# Autodesk Inventor assembly: BevelTo20TSpureGear
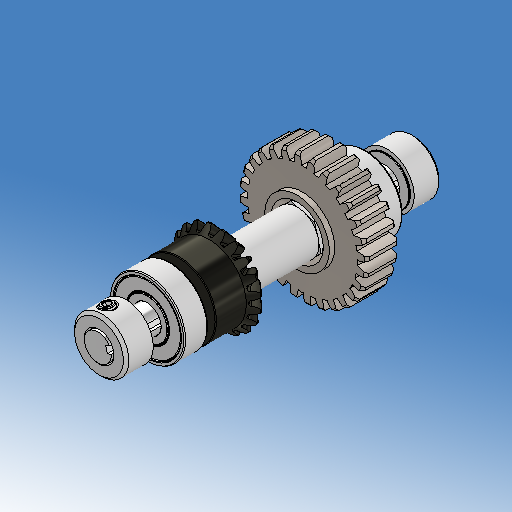
[picture p0: Inventor's stored thumbnail of the model, 512x512]
Saved by Autodesk Inventor 2025 (Build 290162000, 162)
## iProperties
Created: 2024-04-23
Part Number: BevelTo20TSpureGear
Document SubType Name: Assembly
Designer: seene
Author: seene
## Documents named in this file (11)
- C:\Users\seene\OneDrive\SBRT\Robocup Rescue\Drive\v1\BevelTo20TSpureGear.iam
- C:\Users\seene\OneDrive\SBRT\Robocup Rescue\Drive\v1\1439K211_1045 Carbon Steel Keyed Rotary Shaft.ipt
- C:\Users\seene\OneDrive\SBRT\Robocup Rescue\Drive\v1\am-3776 Miter Gear 1.25, 20T, 8mm, 2mm Key Bore.ipt
- C:\Users\seene\OneDrive\SBRT\Robocup Rescue\Drive\v1\am-0588_short 8mm 500 Hex Adapter Shaft 500 long.ipt
- C:\Users\seene\OneDrive\SBRT\Robocup Rescue\Drive\v1\Gears\am-5133 28T 20DP 500hex 375 FW.ipt
- C:\Users\seene\OneDrive\SBRT\Robocup Rescue\Drive\v1\2349K744_Permanently Lubricated Ball Bearing.ipt
- C:\Users\seene\OneDrive\SBRT\Robocup Rescue\Drive\v1\8mKeyyedShaftSpacer_BevelToSpurShaft.ipt
- C:\Users\seene\OneDrive\SBRT\Robocup Rescue\Drive\v1\MachinedKeyStock_BevelToSpur.ipt
- C:\Users\seene\OneDrive\SBRT\Robocup Rescue\Drive\v1\8mmKeyedShaftLongSpacer_BevelToSpurShaft.ipt
- C:\Users\seene\OneDrive\SBRT\Robocup Rescue\Drive\v1\98089A336_18-8 Stainless Steel Round Shim.ipt
- C:\Users\seene\OneDrive\SBRT\Robocup Rescue\Drive\v1\6056N16_Carbon Steel Set Screw Collar.ipt
## Components (14 placed, 10 different names)
1. 1439K211_1045 Carbon Steel Keyed Rotary Shaft:1 — Mate:26, Mate:27, Mate:29, Mate:30, Mate:31, Mate:32, Mate:33, Mate:34, Mate:35, Mate:36, Mate:37, Mate:38, Mate:39, Mate:41
2. am-3776 Miter Gear 1.25, 20T, 8mm, 2mm Key Bore:1 — Mate:19, Flush:8, Mate:22, Flush:9, Flush:10
3. am-0588_short 8mm 500 Hex Adapter Shaft 500 long:1 — Mate:4, Mate:32, Flush:11
4. am-5133 28T 20DP 500hex 375 FW:1 — Mate:4, Mate:25, Mate:33, Flush:11
5. 2349K744_Permanently Lubricated Ball Bearing:1 — Mate:11, Mate:17, Mate:35, Flush:14
6. 2349K744_Permanently Lubricated Ball Bearing:2 — Mate:11, Mate:23, Mate:26, Mate:27, Mate:28, Flush:15
7. 8mKeyyedShaftSpacer_BevelToSpurShaft:1 — Mate:17, Mate:19, Mate:36
8. MachinedKeyStock_BevelToSpur:1 — Flush:8, Mate:30, Mate:31
9. 8mmKeyedShaftLongSpacer_BevelToSpurShaft:1 — Mate:22, Flush:9, Flush:10, Mate:34
10. 98089A336_18-8 Stainless Steel Round Shim:1 — Mate:23, Mate:25, Mate:28, Mate:29
11. 6056N16_Carbon Steel Set Screw Collar:1 — Mate:37, Mate:40
12. 6056N16_Carbon Steel Set Screw Collar:2 — Mate:38, Mate:42
13. 98089A336_18-8 Stainless Steel Round Shim:2 — Mate:39, Flush:14, Mate:40
14. 98089A336_18-8 Stainless Steel Round Shim:3 — Mate:41, Flush:15, Mate:42
## Relationships (30: Mate 24, Flush 6)
- Mate:4: am-0588_short 8mm 500 Hex Adapter Shaft 500 long:1 ↔ am-5133 28T 20DP 500hex 375 FW:1
- Mate:11 (50.8 mm): 2349K744_Permanently Lubricated Ball Bearing:1 ↔ 2349K744_Permanently Lubricated Ball Bearing:2
- Mate:17: 2349K744_Permanently Lubricated Ball Bearing:1 ↔ 8mKeyyedShaftSpacer_BevelToSpurShaft:1
- Mate:19: am-3776 Miter Gear 1.25, 20T, 8mm, 2mm Key Bore:1 ↔ 8mKeyyedShaftSpacer_BevelToSpurShaft:1
- Flush:8: am-3776 Miter Gear 1.25, 20T, 8mm, 2mm Key Bore:1 ↔ MachinedKeyStock_BevelToSpur:1
- Mate:22: am-3776 Miter Gear 1.25, 20T, 8mm, 2mm Key Bore:1 ↔ 8mmKeyedShaftLongSpacer_BevelToSpurShaft:1
- Flush:9: am-3776 Miter Gear 1.25, 20T, 8mm, 2mm Key Bore:1 ↔ 8mmKeyedShaftLongSpacer_BevelToSpurShaft:1
- Flush:10: am-3776 Miter Gear 1.25, 20T, 8mm, 2mm Key Bore:1 ↔ 8mmKeyedShaftLongSpacer_BevelToSpurShaft:1
- Mate:23: 2349K744_Permanently Lubricated Ball Bearing:2 ↔ 98089A336_18-8 Stainless Steel Round Shim:1
- Mate:25: am-5133 28T 20DP 500hex 375 FW:1 ↔ 98089A336_18-8 Stainless Steel Round Shim:1
- Mate:26 (-21.2 mm): 1439K211_1045 Carbon Steel Keyed Rotary Shaft:1 ↔ 2349K744_Permanently Lubricated Ball Bearing:2
- Mate:27: 1439K211_1045 Carbon Steel Keyed Rotary Shaft:1 ↔ 2349K744_Permanently Lubricated Ball Bearing:2
- Mate:28: 2349K744_Permanently Lubricated Ball Bearing:2 ↔ 98089A336_18-8 Stainless Steel Round Shim:1
- Mate:29: 1439K211_1045 Carbon Steel Keyed Rotary Shaft:1 ↔ 98089A336_18-8 Stainless Steel Round Shim:1
- Mate:30: 1439K211_1045 Carbon Steel Keyed Rotary Shaft:1 ↔ MachinedKeyStock_BevelToSpur:1
- Mate:31: 1439K211_1045 Carbon Steel Keyed Rotary Shaft:1 ↔ MachinedKeyStock_BevelToSpur:1
- Mate:32: 1439K211_1045 Carbon Steel Keyed Rotary Shaft:1 ↔ am-0588_short 8mm 500 Hex Adapter Shaft 500 long:1
- Mate:33: 1439K211_1045 Carbon Steel Keyed Rotary Shaft:1 ↔ am-5133 28T 20DP 500hex 375 FW:1
- Flush:11: am-0588_short 8mm 500 Hex Adapter Shaft 500 long:1 ↔ am-5133 28T 20DP 500hex 375 FW:1
- Mate:34: 1439K211_1045 Carbon Steel Keyed Rotary Shaft:1 ↔ 8mmKeyedShaftLongSpacer_BevelToSpurShaft:1
- Mate:35: 1439K211_1045 Carbon Steel Keyed Rotary Shaft:1 ↔ 2349K744_Permanently Lubricated Ball Bearing:1
- Mate:36: 1439K211_1045 Carbon Steel Keyed Rotary Shaft:1 ↔ 8mKeyyedShaftSpacer_BevelToSpurShaft:1
- Mate:37: 1439K211_1045 Carbon Steel Keyed Rotary Shaft:1 ↔ 6056N16_Carbon Steel Set Screw Collar:1
- Mate:38: 1439K211_1045 Carbon Steel Keyed Rotary Shaft:1 ↔ 6056N16_Carbon Steel Set Screw Collar:2
- Mate:39: 1439K211_1045 Carbon Steel Keyed Rotary Shaft:1 ↔ 98089A336_18-8 Stainless Steel Round Shim:2
- Flush:14 (12.7 mm): 2349K744_Permanently Lubricated Ball Bearing:1 ↔ 98089A336_18-8 Stainless Steel Round Shim:2
- Mate:40: 6056N16_Carbon Steel Set Screw Collar:1 ↔ 98089A336_18-8 Stainless Steel Round Shim:2
- Mate:41: 1439K211_1045 Carbon Steel Keyed Rotary Shaft:1 ↔ 98089A336_18-8 Stainless Steel Round Shim:3
- Flush:15 (12.7 mm): 2349K744_Permanently Lubricated Ball Bearing:2 ↔ 98089A336_18-8 Stainless Steel Round Shim:3
- Mate:42: 6056N16_Carbon Steel Set Screw Collar:2 ↔ 98089A336_18-8 Stainless Steel Round Shim:3
